# Autodesk Inventor assembly: gripper2_v5
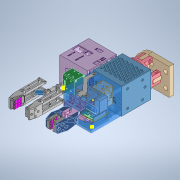
[picture p0: Inventor's stored thumbnail of the model, 180x180]
Saved by Autodesk Inventor 2022 (Build 260153000, 153)
## iProperties
Created: 2022-05-22
Part Number: gripper2_v5
Document SubType Name: Assembly
Designer: kylem
Author: kylem
## Documents named in this file (16)
- C:\Users\kylem\OneDrive\Documents\GitHub\IMML_Contactile_Gripper_Hardware\gripper_v2\gripper2_v5.iam
- C:\Users\kylem\OneDrive\Documents\GitHub\IMML_Contactile_Gripper_Hardware\Gripper_Design_NonCompliant_No_UR5_v3.iam
- C:\Users\kylem\OneDrive\Documents\GitHub\IMML_Contactile_Gripper_Hardware\Contactile_Sensor.ipt
- C:\Users\kylem\OneDrive\Documents\GitHub\IMML_Contactile_Gripper_Hardware\gripper_v2\parallel_bar_short_v1.ipt
- C:\Users\kylem\OneDrive\Documents\GitHub\IMML_Contactile_Gripper_Hardware\gripper_v2\bell_crank_v1.ipt
- C:\Users\kylem\OneDrive\Documents\GitHub\IMML_Contactile_Gripper_Hardware\Motor_XM,H-430_idler.ipt
- C:\Users\kylem\OneDrive\Documents\GitHub\IMML_Contactile_Gripper_Hardware\gripper_v2\base_v1.ipt
- C:\Users\kylem\Downloads\9657K412_Compression Spring.ipt
- C:\Users\kylem\Downloads\5108N177_Music Wire Steel Extension Spring with Loop Ends.ipt
- C:\Users\kylem\OneDrive\Documents\GitHub\IMML_Contactile_Gripper_Hardware\Electronics Box.ipt
- C:\Users\kylem\OneDrive\Documents\GitHub\IMML_Contactile_Gripper_Hardware\gripper_v2\short_link_v2.ipt
- C:\Users\kylem\OneDrive\Documents\GitHub\IMML_Contactile_Gripper_Hardware\gripper_v2\finger_v1.ipt
- C:\Users\kylem\OneDrive\Documents\GitHub\IMML_Contactile_Gripper_Hardware\gripper_v2\parallel_bar_long_no_hole_v2.ipt
- C:\Users\kylem\OneDrive\Documents\GitHub\IMML_Contactile_Gripper_Hardware\gripper_v2\parallel_bar_long_hole_v1.ipt
- C:\Users\kylem\OneDrive\Documents\GitHub\IMML_Contactile_Gripper_Hardware\gripper_v2\link_v4.ipt
- C:\Users\kylem\OneDrive\Documents\GitHub\IMML_Contactile_Gripper_Hardware\gripper_v2\drive_shaft_v4.ipt
## Components (29 placed, 15 different names)
1. Contactile_Sensor:1 — Mate:107, Mate:108, Mate:109
2. parallel_bar_short_v1:1 — Mate:3, Mate:4, Flush:1, Flush:8, Mate:15, Flush:9, Symmetry:1, Mate:101, Mate:102, Mate:149, Mate:154
3. parallel_bar_short_v1:3 — Flush:8, Mate:15, Flush:9, Flush:24, Mate:33, Flush:25, Angle:1, Mate:75, Mate:150, Mate:155
4. Contactile_Sensor:3 — Mate:106, Mate:126, Mate:127, Mate:128
5. parallel_bar_short_v1:5 — Flush:25, Mate:73, Mate:117, Mate:121
6. parallel_bar_short_v1:7 — Flush:24, Mate:33, Symmetry:1, Mate:119, Flush:44, Mate:125, Mate:131, Mate:133, Mate:141
7. Gripper_Design_NonCompliant_No_UR5_v3:1 [sub-assembly] — Angle:1
8. bell_crank_v1:2 — Mate:98, Mate:101, Mate:102, Mate:138, Mate:144, Mate:146, Flush:48
9. Motor_XM,H-430_idler:1 — Mate:73, Mate:78
10. base_v1:1 — Mate:75
11. 9657K412_Compression Spring:1
12. 5108N177_Music Wire Steel Extension Spring with Loop Ends:1
13. Electronics Box:1 — Mate:78
14. short_link_v2:1 — Mate:98, Mate:138, Mate:151
15. finger_v1:1 — Mate:106, Mate:116, Mate:118, Flush:40, Flush:41, Mate:120, Flush:42, Mate:122, Flush:43, Mate:126, Mate:127, Mate:128, Flush:45
16. finger_v1:2 — Mate:107, Mate:108, Mate:109, Mate:147, Mate:148, Flush:45, Mate:152, Mate:153
17. parallel_bar_long_no_hole_v2:1 — Mate:116, Flush:41, Mate:125, Mate:132, Mate:142, Flush:46
18. parallel_bar_long_no_hole_v2:2 — Mate:117, Mate:118, Flush:40, Flush:47
19. parallel_bar_long_hole_v1:1 — Mate:119, Mate:120, Flush:42, Flush:44, Mate:136
20. parallel_bar_long_hole_v1:2 — Mate:121, Mate:122, Flush:43
21. bell_crank_v1:3 — Mate:131, Mate:132, Mate:133, Mate:135, Mate:137, Mate:139, Mate:140, Flush:48
22. short_link_v2:2 — Mate:135, Mate:136, Mate:137
23. link_v4:1 — Mate:139, Mate:140, Mate:143
24. drive_shaft_v4:1 — Mate:141, Mate:142, Mate:143, Mate:145
25. link_v4:2 — Mate:144, Mate:145, Mate:146
26. parallel_bar_long_hole_v1:3 — Mate:148, Mate:150, Flush:47, Flush:50
27. parallel_bar_long_hole_v1:4 — Mate:147, Mate:149, Mate:151, Flush:46, Flush:49
28. parallel_bar_long_no_hole_v2:3 — Mate:153, Flush:50, Mate:155
29. parallel_bar_long_no_hole_v2:4 — Mate:152, Flush:49, Mate:154
## Relationships (70: Mate 50, Flush 18, Angle 1, Symmetry 1)
- Mate:3: parallel_bar_short_v1:1
- Mate:4: parallel_bar_short_v1:1
- Flush:1: parallel_bar_short_v1:1
- Flush:8: parallel_bar_short_v1:1 ↔ parallel_bar_short_v1:3
- Mate:15 (16 mm): parallel_bar_short_v1:1 ↔ parallel_bar_short_v1:3
- Flush:9: parallel_bar_short_v1:1 ↔ parallel_bar_short_v1:3
- [Flush]: parallel_bar_short_v1:5 ↔ parallel_bar_short_v1:7
- [Mate] (16 mm): parallel_bar_short_v1:5 ↔ parallel_bar_short_v1:7
- [Flush]: parallel_bar_short_v1:5 ↔ parallel_bar_short_v1:7
- Flush:24: parallel_bar_short_v1:3 ↔ parallel_bar_short_v1:7
- Mate:33 (30 mm): parallel_bar_short_v1:3 ↔ parallel_bar_short_v1:7
- Flush:25: parallel_bar_short_v1:3 ↔ parallel_bar_short_v1:5
- Angle:1 (0 deg): parallel_bar_short_v1:3 ↔ Gripper_Design_NonCompliant_No_UR5_v3:1
- Symmetry:1: parallel_bar_short_v1:1 ↔ parallel_bar_short_v1:7
- Mate:73 (30.5 mm): parallel_bar_short_v1:5 ↔ Motor_XM,H-430_idler:1
- Mate:75 (16 mm): parallel_bar_short_v1:3 ↔ base_v1:1
- Mate:78: Motor_XM,H-430_idler:1 ↔ Electronics Box:1
- Mate:98: bell_crank_v1:2 ↔ short_link_v2:1
- Mate:101 (-0.5 mm): parallel_bar_short_v1:1 ↔ bell_crank_v1:2
- Mate:102 (-19.5 mm): parallel_bar_short_v1:1 ↔ bell_crank_v1:2
- Mate:106: Contactile_Sensor:3 ↔ finger_v1:1
- Mate:107: Contactile_Sensor:1 ↔ finger_v1:2
- Mate:108: Contactile_Sensor:1 ↔ finger_v1:2
- Mate:109: Contactile_Sensor:1 ↔ finger_v1:2
- Mate:116: finger_v1:1 ↔ parallel_bar_long_no_hole_v2:1
- Mate:117: parallel_bar_short_v1:5 ↔ parallel_bar_long_no_hole_v2:2
- Mate:118: finger_v1:1 ↔ parallel_bar_long_no_hole_v2:2
- Flush:40: finger_v1:1 ↔ parallel_bar_long_no_hole_v2:2
- Flush:41: finger_v1:1 ↔ parallel_bar_long_no_hole_v2:1
- Mate:119: parallel_bar_short_v1:7 ↔ parallel_bar_long_hole_v1:1
- Mate:120: finger_v1:1 ↔ parallel_bar_long_hole_v1:1
- Flush:42: finger_v1:1 ↔ parallel_bar_long_hole_v1:1
- Mate:121: parallel_bar_short_v1:5 ↔ parallel_bar_long_hole_v1:2
- Mate:122: finger_v1:1 ↔ parallel_bar_long_hole_v1:2
- Flush:43: finger_v1:1 ↔ parallel_bar_long_hole_v1:2
- Flush:44: parallel_bar_short_v1:7 ↔ parallel_bar_long_hole_v1:1
- Mate:125: parallel_bar_short_v1:7 ↔ parallel_bar_long_no_hole_v2:1
- Mate:126: Contactile_Sensor:3 ↔ finger_v1:1
- Mate:127: Contactile_Sensor:3 ↔ finger_v1:1
- Mate:128: Contactile_Sensor:3 ↔ finger_v1:1
- Mate:131 (-19.5 mm): parallel_bar_short_v1:7 ↔ bell_crank_v1:3
- Mate:132 (5.75 mm): parallel_bar_long_no_hole_v2:1 ↔ bell_crank_v1:3
- Mate:133 (-0.5 mm): parallel_bar_short_v1:7 ↔ bell_crank_v1:3
- Mate:135: bell_crank_v1:3 ↔ short_link_v2:2
- Mate:136: parallel_bar_long_hole_v1:1 ↔ short_link_v2:2
- Mate:137 (0.2 mm): bell_crank_v1:3 ↔ short_link_v2:2
- Mate:138 (0.2 mm): bell_crank_v1:2 ↔ short_link_v2:1
- Mate:139 (0.2 mm): bell_crank_v1:3 ↔ link_v4:1
- Mate:140: bell_crank_v1:3 ↔ link_v4:1
- Mate:141 (15 mm): parallel_bar_short_v1:7 ↔ drive_shaft_v4:1
- Mate:142 (-13.75 mm): parallel_bar_long_no_hole_v2:1 ↔ drive_shaft_v4:1
- Mate:143: link_v4:1 ↔ drive_shaft_v4:1
- Mate:144: bell_crank_v1:2 ↔ link_v4:2
- Mate:145: drive_shaft_v4:1 ↔ link_v4:2
- Mate:146 (0.2 mm): bell_crank_v1:2 ↔ link_v4:2
- Mate:147: finger_v1:2 ↔ parallel_bar_long_hole_v1:4
- Mate:148: finger_v1:2 ↔ parallel_bar_long_hole_v1:3
- Mate:149: parallel_bar_short_v1:1 ↔ parallel_bar_long_hole_v1:4
- Mate:150: parallel_bar_short_v1:3 ↔ parallel_bar_long_hole_v1:3
- Mate:151: short_link_v2:1 ↔ parallel_bar_long_hole_v1:4
- Flush:45: finger_v1:1 ↔ finger_v1:2
- Flush:46: parallel_bar_long_no_hole_v2:1 ↔ parallel_bar_long_hole_v1:4
- Flush:47: parallel_bar_long_no_hole_v2:2 ↔ parallel_bar_long_hole_v1:3
- Mate:152: finger_v1:2 ↔ parallel_bar_long_no_hole_v2:4
- Mate:153: finger_v1:2 ↔ parallel_bar_long_no_hole_v2:3
- Flush:48: bell_crank_v1:2 ↔ bell_crank_v1:3
- Flush:49: parallel_bar_long_hole_v1:4 ↔ parallel_bar_long_no_hole_v2:4
- Flush:50: parallel_bar_long_hole_v1:3 ↔ parallel_bar_long_no_hole_v2:3
- Mate:154: parallel_bar_short_v1:1 ↔ parallel_bar_long_no_hole_v2:4
- Mate:155: parallel_bar_short_v1:3 ↔ parallel_bar_long_no_hole_v2:3
## Named parameters: d32_d22 = 16 mm, d33_d23 = 0 mm, d55_d21 = 0 mm
